# Autodesk Inventor assembly: LegHandleDrawing
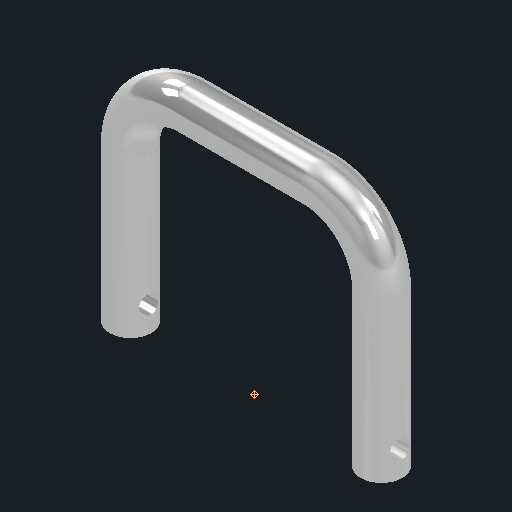
[picture p0: Inventor's stored thumbnail of the model, 512x512]
Saved by Autodesk Inventor 2025.2 (Build 292293000, 293)
## iProperties
Created: 2025-10-20
Part Number: LegHandleDrawing
Document SubType Name: Assembly
Designer: valer
Author: valer
## Documents named in this file (2)
- C:\Users\valer\Desktop\str1ker\cad\LegHandleDrawing.iam
- C:\Users\valer\Desktop\str1ker\cad\LegHandle.iam
## Components (1 placed, 1 different names)
1. LegHandle:1 [sub-assembly] — Mate:1, Mate:2, Mate:3, Mate:4
## Relationships (4: Mate 4)
- Mate:1: LegHandle:1
- Mate:2: LegHandle:1
- Mate:3: LegHandle:1
- Mate:4: LegHandle:1
